# Autodesk Inventor assembly: Wheel Orientation
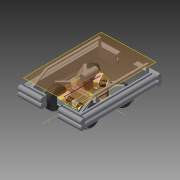
[picture p0: Inventor's stored thumbnail of the model, 180x180]
Saved by Autodesk Inventor 2015 (Build 190159000, 159)
## iProperties
Created: 2016-01-19
Part Number: Wheel Orientation
Document SubType Name: Assembly
Designer: sethbattis
Author: sethbattis
## Documents named in this file (9)
- \\area51\team3566\cad\FRC 2016\Space Claims.iam
- \\area51\team3566\cad\FRC 2016\Wheelbase.ipt
- \\area51\team3566\cad\FRC 2016\Basic Frame.ipt
- \\area51\team3566\cad\FRC 2016\Roll Bar.ipt
- \\area51\team3566\cad\FRC 2016\Snow Blower Tire with Gear Box and Mini-CIM.iam
- \\area51\team3566\cad\FRC 2016\Snow Blower Tire with Gear Box and Mini-CIM_MIR.iam
- \\area51\team3566\cad\FRC 2016\Center Truss.ipt
- \\area51\team3566\cad\FRC 2016\Side Bumper.ipt
- \\area51\team3566\cad\FRC 2016\Extension Grappel.ipt
## Components (12 placed, 8 different names)
1. Basic Frame:1 — Flush:1, Rigid:1, Mate:12, Flush:11, Flush:12, Flush:13, Flush:14, Flush:15, Rigid:2, Rigid:3, Mate:13, Flush:16, Flush:17, Mate:14, Flush:18, Flush:19, Tangent:1
2. Wheelbase:1 — Flush:1, Rigid:1, Rotational:1, Rotational:2, Rotational:3, Rotational:4, Angle:1
3. Center Truss:1 — Rigid:2, Rigid:3
4. Extension Grappel:1 — Tangent:1
5. Side Bumper:2 — Mate:14, Flush:18, Flush:19
6. Side Bumper:1 — Mate:13, Flush:16, Flush:17
7. Roll Bar:1 — Flush:12, Flush:13, Flush:15
8. Roll Bar:2 — Mate:12, Flush:11, Flush:14
9. Snow Blower Tire with Gear Box and Mini-CIM:1 [sub-assembly] — Rotational:1
10. Snow Blower Tire with Gear Box and Mini-CIM:2 [sub-assembly] — Rotational:2
11. Snow Blower Tire with Gear Box and Mini-CIM_MIR:1 [sub-assembly] — Rotational:4, Angle:1
12. Snow Blower Tire with Gear Box and Mini-CIM_MIR:2 [sub-assembly] — Rotational:3
## Relationships (22: Flush 10, RevoluteJoint 4, WeldJoint 3, Mate 3, Angle 1, Tangent 1)
- Flush:1: Basic Frame:1 ↔ Wheelbase:1
- Rigid:1 [WeldJoint]: Basic Frame:1 ↔ Wheelbase:1
- Mate:12: Basic Frame:1 ↔ Roll Bar:2
- Flush:11: Basic Frame:1 ↔ Roll Bar:2
- Flush:12: Basic Frame:1 ↔ Roll Bar:1
- Flush:13: Basic Frame:1 ↔ Roll Bar:1
- Flush:14: Basic Frame:1 ↔ Roll Bar:2
- Flush:15: Basic Frame:1 ↔ Roll Bar:1
- Rotational:1 [RevoluteJoint]: Wheelbase:1 ↔ Snow Blower Tire with Gear Box and Mini-CIM:1
- Rotational:2 [RevoluteJoint]: Wheelbase:1 ↔ Snow Blower Tire with Gear Box and Mini-CIM:2
- Rotational:3 [RevoluteJoint]: Wheelbase:1 ↔ Snow Blower Tire with Gear Box and Mini-CIM_MIR:2
- Rotational:4 [RevoluteJoint]: Wheelbase:1 ↔ Snow Blower Tire with Gear Box and Mini-CIM_MIR:1
- Angle:1 (45 deg): Wheelbase:1 ↔ Snow Blower Tire with Gear Box and Mini-CIM_MIR:1
- Rigid:2 [WeldJoint]: Basic Frame:1 ↔ Center Truss:1
- Rigid:3 [WeldJoint]: Basic Frame:1 ↔ Center Truss:1
- Mate:13: Basic Frame:1 ↔ Side Bumper:1
- Flush:16: Basic Frame:1 ↔ Side Bumper:1
- Flush:17: Basic Frame:1 ↔ Side Bumper:1
- Mate:14: Basic Frame:1 ↔ Side Bumper:2
- Flush:18: Basic Frame:1 ↔ Side Bumper:2
- Flush:19: Basic Frame:1 ↔ Side Bumper:2
- Tangent:1: Basic Frame:1 ↔ Extension Grappel:1
